# Autodesk Inventor assembly: Application_OpenFiberCoupling
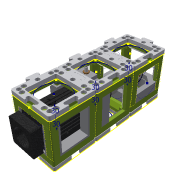
[picture p0: Inventor's stored thumbnail of the model, 180x180]
Saved by Autodesk Inventor 2019.4 (Build 234330000, 330)
## iProperties
Created: 2021-08-13
Part Number: Application_OpenFiberCoupling
Document SubType Name: Assembly
Designer: diederichbenedict
Author: diederichbenedict
## Documents named in this file (8)
- C:\Users\diederichbenedict\Dropbox\Dokumente\Promotion\PROJECTS\UC2\02_CAD\INVENTOR\uc2_v3\Application_OpenFiberCoupling.iam
- C:\Users\diederichbenedict\Dropbox\Dokumente\Promotion\PROJECTS\UC2\02_CAD\INVENTOR\uc2_v3\Assembly_Cube_Laser_Block_v3.iam
- C:\Users\diederichbenedict\Dropbox\Dokumente\Promotion\PROJECTS\UC2\02_CAD\INVENTOR\uc2_v3\Assembly_Cube_Flexuremanipulator_zonly_v3.iam
- C:\Users\diederichbenedict\Dropbox\Dokumente\Promotion\PROJECTS\UC2\02_CAD\INVENTOR\uc2_v3\Assembly_Cube_Flexuremanipulator_v3.iam
- C:\Users\diederichbenedict\Dropbox\Dokumente\Promotion\PROJECTS\UC2\02_CAD\INVENTOR\uc2_v3\10_Base_puzzle_v3.ipt
- C:\Users\diederichbenedict\Dropbox\Dokumente\Promotion\PROJECTS\UC2\02_CAD\INVENTOR\uc2_v3\00_objectivelens_10x.ipt
- C:\Users\diederichbenedict\Downloads\00_F6SSN2P-Step.ipt
- C:\Users\diederichbenedict\Downloads\00_F6SS088-Step.ipt
## Components (12 placed, 7 different names)
1. Assembly_Cube_Laser_Block_v3:1 [sub-assembly] — Insert:1, Angle:4
2. Assembly_Cube_Flexuremanipulator_v3:1 [sub-assembly] — Insert:2, Angle:2, Insert:4
3. 00_objectivelens_10x:1 — Insert:4
4. 00_F6SSN2P-Step:1 — Insert:7
5. 00_F6SS088-Step:1
6. Assembly_Cube_Flexuremanipulator_zonly_v3:1 [sub-assembly] — Insert:6, Angle:5, Insert:7
7. 10_Base_puzzle_v3:1 — Mate:1, Insert:6, Angle:5
8. 10_Base_puzzle_v3:2 — Insert:2, Angle:2, Angle:4
9. 10_Base_puzzle_v3:3 — Insert:1
10. 10_Base_puzzle_v3:4
11. 10_Base_puzzle_v3:5
12. 10_Base_puzzle_v3:6
## Component patterns: (2 elements), (3 elements, first: 10_Base_puzzle_v3:1), Component Pattern 1:2 (3 elements)
## Relationships (10: Insert 6, Angle 3, Mate 1)
- Mate:1: 10_Base_puzzle_v3:1
- Insert:1: Assembly_Cube_Laser_Block_v3:1 ↔ 10_Base_puzzle_v3:3
- Insert:2: Assembly_Cube_Flexuremanipulator_v3:1 ↔ 10_Base_puzzle_v3:2
- Angle:2 (0 deg): Assembly_Cube_Flexuremanipulator_v3:1 ↔ 10_Base_puzzle_v3:2
- Angle:4 (0 deg): Assembly_Cube_Laser_Block_v3:1 ↔ 10_Base_puzzle_v3:2
- Insert:4: Assembly_Cube_Flexuremanipulator_v3:1 ↔ 00_objectivelens_10x:1
- [Insert] (-5 mm): 00_F6SSN2P-Step:1 ↔ 00_F6SS088-Step:1
- Insert:6: Assembly_Cube_Flexuremanipulator_zonly_v3:1 ↔ 10_Base_puzzle_v3:1
- Angle:5 (0 deg): Assembly_Cube_Flexuremanipulator_zonly_v3:1 ↔ 10_Base_puzzle_v3:1
- Insert:7: 00_F6SSN2P-Step:1 ↔ Assembly_Cube_Flexuremanipulator_zonly_v3:1
## Named parameters: d17_d13 = -5 mm
